# Autodesk Inventor assembly: RobotPallet
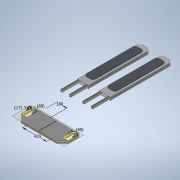
[picture p0: Inventor's stored thumbnail of the model, 180x180]
Saved by Autodesk Inventor 2022 (Build 260153000, 153)
## iProperties
Created: 2021-09-10
Part Number: RobotPallet
Material: Generic
Document SubType Name: Assembly
Designer: Andres
Author: Andres
## Documents named in this file (5)
- C:\Users\andre\Documents\2021-2\pdm\RobotPallet\RobotPallet.iam
- C:\Users\andre\Documents\2021-2\pdm\RobotPallet\Estructura Inferior.iam
- C:\Users\andre\Documents\2021-2\pdm\RobotPallet\Horquillas\Horquilla.iam
- C:\Users\andre\Documents\2021-2\pdm\RobotPallet\plancah base.ipt
- C:\Users\andre\Documents\2021-2\pdm\RobotPallet\apoyo\apoyo2.ipt
## Components (8 placed, 4 different names)
1. Estructura Inferior:1 [sub-assembly] — Flush:1
2. Horquilla:1 [sub-assembly]
3. Horquilla:2 [sub-assembly]
4. planchabase:1 — Flush:1, Nivelación:2, Coincidencia:1, Coincidencia:2, Coincidencia:3, Coincidencia:4
5. apoyo2:1 — Coincidencia:1
6. apoyo2:2 — Coincidencia:2
7. apoyo2:3 — Coincidencia:3
8. apoyo2:4 — Coincidencia:4
## Relationships (6: Mate 4, Flush 2)
- Flush:1: Estructura Inferior:1 ↔ planchabase:1
- Nivelación:2 [Flush]: planchabase:1
- Coincidencia:1 [Mate]: planchabase:1 ↔ apoyo2:1
- Coincidencia:2 [Mate]: planchabase:1 ↔ apoyo2:2
- Coincidencia:3 [Mate]: planchabase:1 ↔ apoyo2:3
- Coincidencia:4 [Mate]: planchabase:1 ↔ apoyo2:4
